# Autodesk Inventor assembly: Rahmen
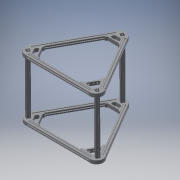
[picture p0: Inventor's stored thumbnail of the model, 180x180]
Saved by Autodesk Inventor 2019 (Build 230136000, 136)
## iProperties
Created: 2018-08-19
Part Number: Rahmen
Document SubType Name: Assembly
Designer: Julia
Author: Julia
## Documents named in this file (3)
- C:\Users\Julia\Documents\Inventor\3d_Drucker_v02\Rahmen.iam
- C:\Users\Julia\Documents\Inventor\3d_Drucker_v02\Rahmen_Dreieck.iam
- C:\Users\Julia\Documents\Inventor\3d_Drucker_v02\Rahmen_Alu_Profil_Dreieck_laengs.ipt
## Components (5 placed, 2 different names)
1. Rahmen_Dreieck:1 [sub-assembly] — Mate:7, Mate:8, Flush:4, Flush:5, Flush:6, Mate:9, Mate:10, Flush:7, Mate:11
2. Rahmen_Dreieck:2 [sub-assembly] — Mate:1, Mate:2, Flush:1, Mate:3, Mate:4, Flush:2, Mate:5, Mate:6, Flush:3
3. Rahmen_Alu_Profil_Dreieck_laengs:1 — Mate:1, Mate:2, Flush:1, Mate:7, Mate:8, Flush:4
4. Rahmen_Alu_Profil_Dreieck_laengs:2 — Mate:3, Mate:4, Flush:2, Flush:6, Mate:9, Mate:10
5. Rahmen_Alu_Profil_Dreieck_laengs:3 — Mate:5, Mate:6, Flush:3, Flush:5, Flush:7, Mate:11
## Relationships (18: Mate 11, Flush 7)
- Mate:1: Rahmen_Dreieck:2 ↔ Rahmen_Alu_Profil_Dreieck_laengs:1
- Mate:2: Rahmen_Dreieck:2 ↔ Rahmen_Alu_Profil_Dreieck_laengs:1
- Flush:1: Rahmen_Dreieck:2 ↔ Rahmen_Alu_Profil_Dreieck_laengs:1
- Mate:3: Rahmen_Dreieck:2 ↔ Rahmen_Alu_Profil_Dreieck_laengs:2
- Mate:4: Rahmen_Dreieck:2 ↔ Rahmen_Alu_Profil_Dreieck_laengs:2
- Flush:2: Rahmen_Dreieck:2 ↔ Rahmen_Alu_Profil_Dreieck_laengs:2
- Mate:5: Rahmen_Dreieck:2 ↔ Rahmen_Alu_Profil_Dreieck_laengs:3
- Mate:6: Rahmen_Dreieck:2 ↔ Rahmen_Alu_Profil_Dreieck_laengs:3
- Flush:3: Rahmen_Dreieck:2 ↔ Rahmen_Alu_Profil_Dreieck_laengs:3
- Mate:7: Rahmen_Dreieck:1 ↔ Rahmen_Alu_Profil_Dreieck_laengs:1
- Mate:8: Rahmen_Dreieck:1 ↔ Rahmen_Alu_Profil_Dreieck_laengs:1
- Flush:4: Rahmen_Dreieck:1 ↔ Rahmen_Alu_Profil_Dreieck_laengs:1
- Flush:5: Rahmen_Dreieck:1 ↔ Rahmen_Alu_Profil_Dreieck_laengs:3
- Flush:6: Rahmen_Dreieck:1 ↔ Rahmen_Alu_Profil_Dreieck_laengs:2
- Mate:9: Rahmen_Dreieck:1 ↔ Rahmen_Alu_Profil_Dreieck_laengs:2
- Mate:10: Rahmen_Dreieck:1 ↔ Rahmen_Alu_Profil_Dreieck_laengs:2
- Flush:7: Rahmen_Dreieck:1 ↔ Rahmen_Alu_Profil_Dreieck_laengs:3
- Mate:11: Rahmen_Dreieck:1 ↔ Rahmen_Alu_Profil_Dreieck_laengs:3
